# Autodesk Inventor assembly: WheelNSmallChainGear-sandwich
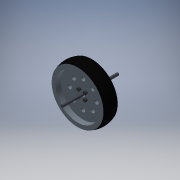
[picture p0: Inventor's stored thumbnail of the model, 180x180]
Saved by Autodesk Inventor 2016 (Build 200138000, 138)
## iProperties
Created: 2015-08-30
Part Number: WheelNSmallChainGear-sandwich
Document SubType Name: Assembly
Designer: Tim
Author: Tim
## Documents named in this file (7)
- C:\Users\Tim\Documents\GitHub\phi_robotics\3d-models\FTC_Tetrix_KOP_Block_Party\Tim Bloot Designs\WheelNSmallChainGear-sandwich.iam
- C:\Users\Tim\Documents\GitHub\phi_robotics\3d-models\FTC_Tetrix_KOP_Block_Party\Tetrix_Kit_FTC\Autodesk Inventor Files\tetrix_wheel.ipt
- C:\Users\Tim\Documents\GitHub\phi_robotics\3d-models\FTC_Tetrix_KOP_Block_Party\Tetrix_Kit_FTC\Autodesk Inventor Files\tetrix_axle_lock.iam
- C:\Users\Tim\Documents\GitHub\phi_robotics\3d-models\FTC_Tetrix_KOP_Block_Party\Tetrix_Kit_FTC\Autodesk Inventor Files\tetrix_axle_spacer_mount.ipt
- C:\Users\Tim\Documents\GitHub\phi_robotics\3d-models\FTC_Tetrix_KOP_Block_Party\Tetrix_Kit_FTC\Autodesk Inventor Files\tetrix_axle.ipt
- C:\Users\Tim\Documents\GitHub\phi_robotics\3d-models\FTC_Tetrix_KOP_Block_Party\Tetrix_Kit_FTC\Autodesk Inventor Files\tetrix_chain_gear-16t.ipt
- C:\Users\Tim\Documents\GitHub\phi_robotics\3d-models\FTC_Tetrix_KOP_Block_Party\Tetrix_Kit_FTC\Autodesk Inventor Files\tetrix_motor_screw-short.ipt
## Components (9 placed, 6 different names)
1. tetrix_wheel:1 — Rigid:1, Rotational:1, Rotational:2, Rotational:3, Rotational:4
2. tetrix_axle_spacer_mount:1 — Rigid:1, Rigid:6, Rigid:8
3. tetrix_axle:1 — Rigid:8
4. tetrix_axle_lock:2 [sub-assembly] — Rigid:7
5. tetrix_chain_gear-16t:1 — Rigid:6, Rigid:7
6. tetrix_motor_screw-short:1 — Rotational:4
7. tetrix_motor_screw-short:2 — Rotational:3
8. tetrix_motor_screw-short:3 — Rotational:2
9. tetrix_motor_screw-short:4 — Rotational:1
## Relationships (8: WeldJoint 4, RevoluteJoint 4)
- Rigid:1 [WeldJoint]: tetrix_wheel:1 ↔ tetrix_axle_spacer_mount:1
- Rigid:6 [WeldJoint]: tetrix_axle_spacer_mount:1 ↔ tetrix_chain_gear-16t:1
- Rigid:7 [WeldJoint]: tetrix_axle_lock:2 ↔ tetrix_chain_gear-16t:1
- Rotational:1 [RevoluteJoint]: tetrix_wheel:1 ↔ tetrix_motor_screw-short:4
- Rotational:2 [RevoluteJoint]: tetrix_wheel:1 ↔ tetrix_motor_screw-short:3
- Rotational:3 [RevoluteJoint]: tetrix_wheel:1 ↔ tetrix_motor_screw-short:2
- Rotational:4 [RevoluteJoint]: tetrix_wheel:1 ↔ tetrix_motor_screw-short:1
- Rigid:8 [WeldJoint]: tetrix_axle_spacer_mount:1 ↔ tetrix_axle:1
